# Autodesk Inventor assembly: Functioning elevator (shaft)
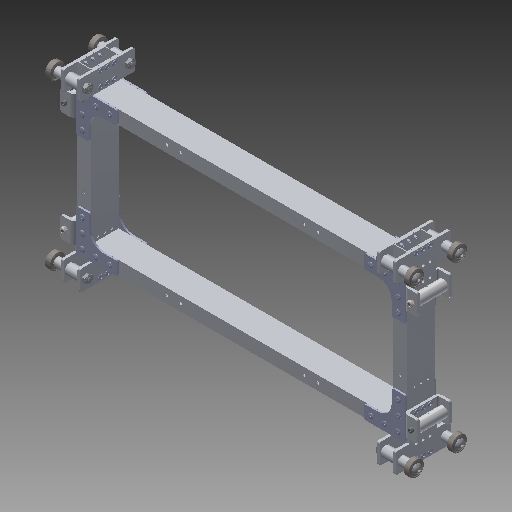
[picture p0: Inventor's stored thumbnail of the model, 512x512]
Saved by Autodesk Inventor 2019 (Build 230136000, 136)
## iProperties
Created: 2019-01-17
Part Number: Functioning elevator (shaft)
Document SubType Name: Assembly
Designer: josh
Mass: 2509.64 g
Surface Area: 8448.9 cm^2
Volume: 929.497 cm^3
Density: 2.7 g/cm^3
Author: josh
## Documents named in this file (5)
- C:\Users\josh\Desktop\Epsilon elavator lift\Functioning elevator (shaft).iam
- C:\Users\josh\Desktop\Epsilon elavator lift\Functioning elevator parts\Example Bearing Tube.ipt
- C:\Users\josh\Desktop\Epsilon elavator lift\Functioning elevator parts\Example Single Corner Bearing Assembly R2.iam
- C:\Users\josh\Desktop\Epsilon elavator lift\Functioning elevator parts\Example Cross Carriage Tube.ipt
- C:\Users\josh\Desktop\Epsilon elavator lift\Functioning elevator parts\am-3860 90 Gusset with Rivets.iam
## Components (16 placed, 4 different names)
1. Example Bearing Tube:1 — Mate:6, Mate:7, Flush:6, Flush:7, Mate:8, Mate:9, Flush:8, Mate:11, Flush:18, Flush:21, Mate:21, Flush:22
2. Example Bearing Tube:2 — Mate:1, Mate:2, Mate:3, Flush:3, Flush:9, Mate:13, Flush:10, Mate:14, Mate:15, Flush:12, Flush:14, Mate:16, Flush:16, Mate:18, Mate:19, Flush:17
3. Example Single Corner Bearing Assembly R2:1 [sub-assembly] — Mate:7, Flush:6, Flush:7, Mate:10
4. Example Single Corner Bearing Assembly R2:2 [sub-assembly] — Mate:21, Mate:22, Flush:22
5. Example Single Corner Bearing Assembly R2:3 [sub-assembly] — Mate:1, Mate:2, Mate:3, Mate:12
6. Example Single Corner Bearing Assembly R2:4 [sub-assembly] — Mate:19, Mate:20, Flush:17
7. Example Cross Carriage Tube:1 — Flush:13, Flush:15, Mate:17, Mate:18, Mate:20, Flush:19, Flush:20, Mate:22
8. Example Cross Carriage Tube:2 — Flush:1, Flush:4, Mate:4, Flush:5, Mate:5, Mate:6, Flush:11, Mate:15
9. am-3860 90 Gusset with Rivets:1 [sub-assembly] — Flush:18, Flush:19
10. am-3860 90 Gusset with Rivets:2 [sub-assembly] — Flush:20, Flush:21
11. am-3860 90 Gusset with Rivets:3 [sub-assembly] — Flush:14, Flush:15, Mate:16, Mate:17, Flush:16
12. am-3860 90 Gusset with Rivets:4 [sub-assembly] — Flush:10, Flush:11, Mate:14
13. am-3860 90 Gusset with Rivets:5 [sub-assembly] — Flush:8, Mate:10, Mate:11
14. am-3860 90 Gusset with Rivets:6 [sub-assembly] — Flush:5, Mate:5, Mate:8, Mate:9
15. am-3860 90 Gusset with Rivets:7 [sub-assembly] — Flush:1, Flush:3, Flush:4, Mate:4, Mate:12, Flush:9, Mate:13
16. am-3860 90 Gusset with Rivets:8 [sub-assembly] — Flush:12, Flush:13
## Relationships (43: Mate 22, Flush 21)
- Flush:1: Example Cross Carriage Tube:2 ↔ am-3860 90 Gusset with Rivets:7
- Mate:1: Example Bearing Tube:2 ↔ Example Single Corner Bearing Assembly R2:3
- Mate:2: Example Bearing Tube:2 ↔ Example Single Corner Bearing Assembly R2:3
- Mate:3: Example Bearing Tube:2 ↔ Example Single Corner Bearing Assembly R2:3
- Flush:3: Example Bearing Tube:2 ↔ am-3860 90 Gusset with Rivets:7
- Flush:4: Example Cross Carriage Tube:2 ↔ am-3860 90 Gusset with Rivets:7
- Mate:4: Example Cross Carriage Tube:2 ↔ am-3860 90 Gusset with Rivets:7
- Flush:5: Example Cross Carriage Tube:2 ↔ am-3860 90 Gusset with Rivets:6
- Mate:5: Example Cross Carriage Tube:2 ↔ am-3860 90 Gusset with Rivets:6
- Mate:6: Example Bearing Tube:1 ↔ Example Cross Carriage Tube:2
- Mate:7: Example Bearing Tube:1 ↔ Example Single Corner Bearing Assembly R2:1
- Flush:6: Example Bearing Tube:1 ↔ Example Single Corner Bearing Assembly R2:1
- Flush:7: Example Bearing Tube:1 ↔ Example Single Corner Bearing Assembly R2:1
- Mate:8: Example Bearing Tube:1 ↔ am-3860 90 Gusset with Rivets:6
- Mate:9: Example Bearing Tube:1 ↔ am-3860 90 Gusset with Rivets:6
- Flush:8: Example Bearing Tube:1 ↔ am-3860 90 Gusset with Rivets:5
- Mate:10: Example Single Corner Bearing Assembly R2:1 ↔ am-3860 90 Gusset with Rivets:5
- Mate:11: Example Bearing Tube:1 ↔ am-3860 90 Gusset with Rivets:5
- Mate:12: Example Single Corner Bearing Assembly R2:3 ↔ am-3860 90 Gusset with Rivets:7
- Flush:9: Example Bearing Tube:2 ↔ am-3860 90 Gusset with Rivets:7
- Mate:13: Example Bearing Tube:2 ↔ am-3860 90 Gusset with Rivets:7
- Flush:10: Example Bearing Tube:2 ↔ am-3860 90 Gusset with Rivets:4
- Flush:11: Example Cross Carriage Tube:2 ↔ am-3860 90 Gusset with Rivets:4
- Mate:14: Example Bearing Tube:2 ↔ am-3860 90 Gusset with Rivets:4
- Mate:15: Example Bearing Tube:2 ↔ Example Cross Carriage Tube:2
- Flush:12: Example Bearing Tube:2 ↔ am-3860 90 Gusset with Rivets:8
- Flush:13: Example Cross Carriage Tube:1 ↔ am-3860 90 Gusset with Rivets:8
- Flush:14: Example Bearing Tube:2 ↔ am-3860 90 Gusset with Rivets:3
- Flush:15: Example Cross Carriage Tube:1 ↔ am-3860 90 Gusset with Rivets:3
- Mate:16: Example Bearing Tube:2 ↔ am-3860 90 Gusset with Rivets:3
- Mate:17: Example Cross Carriage Tube:1 ↔ am-3860 90 Gusset with Rivets:3
- Flush:16: Example Bearing Tube:2 ↔ am-3860 90 Gusset with Rivets:3
- Mate:18: Example Bearing Tube:2 ↔ Example Cross Carriage Tube:1
- Mate:19: Example Bearing Tube:2 ↔ Example Single Corner Bearing Assembly R2:4
- Mate:20: Example Single Corner Bearing Assembly R2:4 ↔ Example Cross Carriage Tube:1
- Flush:17: Example Bearing Tube:2 ↔ Example Single Corner Bearing Assembly R2:4
- Flush:18: Example Bearing Tube:1 ↔ am-3860 90 Gusset with Rivets:1
- Flush:19: Example Cross Carriage Tube:1 ↔ am-3860 90 Gusset with Rivets:1
- Flush:20: Example Cross Carriage Tube:1 ↔ am-3860 90 Gusset with Rivets:2
- Flush:21: Example Bearing Tube:1 ↔ am-3860 90 Gusset with Rivets:2
- Mate:21: Example Bearing Tube:1 ↔ Example Single Corner Bearing Assembly R2:2
- Mate:22: Example Single Corner Bearing Assembly R2:2 ↔ Example Cross Carriage Tube:1
- Flush:22: Example Bearing Tube:1 ↔ Example Single Corner Bearing Assembly R2:2
